# Autodesk Inventor assembly: base mg996r 3mm frame with axis
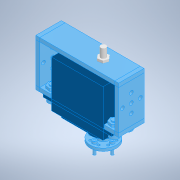
[picture p0: Inventor's stored thumbnail of the model, 180x180]
Saved by Autodesk Inventor 2021.4 (Build 254397000, 397)
## iProperties
Created: 2022-07-09
Part Number: base mg996r 3mm frame with axis
Document SubType Name: Assembly
Designer: isamu
Author: isamu
## Documents named in this file (5)
- D:\personal_projects\robot\inventor\2021\base mg996r 3mm frame with axis.iam
- D:\personal_projects\robot\inventor\2021\base mg996r 3mm frame.iam
- D:\personal_projects\robot\exports\screws\m4x12.ipt
- D:\personal_projects\robot\exports\screws\m4 nuts.ipt
- D:\personal_projects\robot\exports\frames\servo frame mg996r.ipt
## Components (4 placed, 4 different names)
1. base mg996r 3mm frame:1 [sub-assembly] — Insert:1, Insert:2, Mate:1, Mate:3
2. m4x12:1 — Insert:1
3. m4 nuts:1 — Insert:2
4. servo frame mg996r:1 — Mate:1, Mate:3
## Relationships (4: Insert 2, Mate 2)
- Insert:1: base mg996r 3mm frame:1 ↔ m4x12:1
- Insert:2: base mg996r 3mm frame:1 ↔ m4 nuts:1
- Mate:1: base mg996r 3mm frame:1 ↔ servo frame mg996r:1
- Mate:3: base mg996r 3mm frame:1 ↔ servo frame mg996r:1
